# Autodesk Inventor assembly: shaft extender
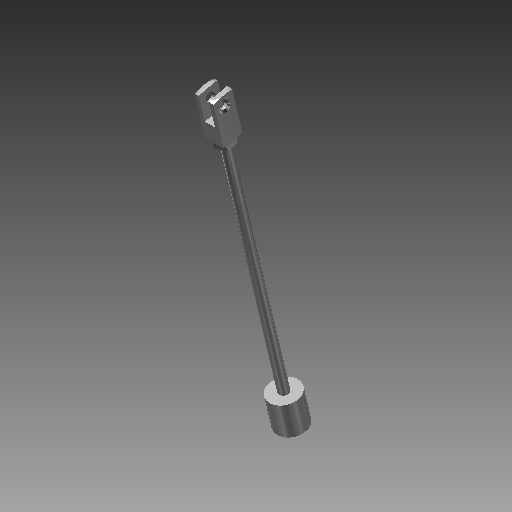
[picture p0: Inventor's stored thumbnail of the model, 512x512]
Saved by Autodesk Inventor 2017 (Build 210142000, 142)
## iProperties
Created: 2016-11-06
Part Number: shaft extender
Document SubType Name: Assembly
Designer: gus
Mass: 15.1397 g
Surface Area: 80.3706 cm^2
Volume: 15.1397 cm^3
Density: 1 g/cm^3
Author: gus
## Documents named in this file (4)
- C:\Users\Thariq\Documents\GitHub\bps-bunnybots2016-cad\bps-bunnybots2016-cad\Bunnybot-Night_Fury\15102898-16-A-0000\15102898-16-A-0900\Imported Components\AIS2015\shaft extender.iam
- C:\Users\Thariq\Documents\GitHub\bps-bunnybots2016-cad\bps-bunnybots2016-cad\Bunnybot-Night_Fury\15102898-16-A-0000\15102898-16-A-0900\Imported Components\AIS2015\C-045-DP0_rod.ipt
- C:\Users\Thariq\Documents\GitHub\bps-bunnybots2016-cad\bps-bunnybots2016-cad\Bunnybot-Night_Fury\15102898-16-A-0000\15102898-16-A-0900\Imported Components\AIS2015\D-14055.ipt
- C:\Users\Thariq\Documents\GitHub\bps-bunnybots2016-cad\bps-bunnybots2016-cad\Bunnybot-Night_Fury\15102898-16-A-0000\15102898-16-A-0900\Imported Components\AIS2015\D-344.ipt
## Components (3 placed, 3 different names)
1. C-045-DP0_rod:1
2. D-14055:1
3. D-344:1
## Relationships (4: Mate 4)
- [Mate]: C-045-DP0_rod:1 ↔ D-14055:1
- [Mate]: C-045-DP0_rod:1 ↔ D-344:1
- [Mate]: C-045-DP0_rod:1 ↔ D-344:1
- [Mate]: D-14055:1 ↔ D-344:1
